# Autodesk Inventor assembly: 1. Prototype Plate Assembly
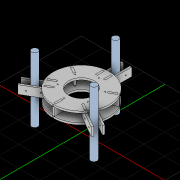
[picture p0: Inventor's stored thumbnail of the model, 180x180]
Saved by Autodesk Inventor 2020.1 (Build 241239000, 239)
## iProperties
Created: 2019-08-27
Part Number: 1. Prototype Plate Assembly
Document SubType Name: Assembly
Designer: Oliver Frolovs
Mass: 1152 g
Surface Area: 3223.44 cm^2
Volume: 1152 cm^3
Density: 1 g/cm^3
Author: Oliver Frolovs
## Documents named in this file (6)
- C:\Users\of12343\Documents\Projects\prototype-plate\1. Prototype Plate Assembly.iam
- C:\Users\of12343\Documents\Projects\prototype-plate\Prototype Plate Base.ipt
- C:\Users\of12343\Documents\Projects\prototype-plate\Inner Rib.ipt
- C:\Users\of12343\Documents\Projects\prototype-plate\0. All Parameters.ipt
- C:\Users\of12343\Documents\Projects\prototype-plate\Outer Rib.ipt
- C:\Users\of12343\Documents\Projects\prototype-plate\Locate Rig Columns.ipt
## Components (12 placed, 4 different names)
1. Prototype Plate Base:1 — Rigid:3, Rigid:4, Rigid:5, Rigid:6
2. Prototype Plate Base:2 — Rigid:4
3. Locate Rig Columns:1 — Flush:1
4. Inner Rib — Rigid:3
5. Inner Rib:2
6. Inner Rib:3
7. Outer Rib:1 — Rigid:5
8. Outer Rib:2 — Rigid:6
9. Outer Rib:3
10. Outer Rib:4
11. Outer Rib:5
12. Outer Rib:6
## Component patterns: Inner Ribs (3 elements), Outer Ribs (3 elements)
## Relationships (5: WeldJoint 4, Flush 1)
- Rigid:3 [WeldJoint]: Prototype Plate Base:1 ↔ Inner Rib
- Rigid:4 [WeldJoint] (40 mm): Prototype Plate Base:1 ↔ Prototype Plate Base:2
- Rigid:5 [WeldJoint]: Prototype Plate Base:1 ↔ Outer Rib:1
- Rigid:6 [WeldJoint]: Prototype Plate Base:1 ↔ Outer Rib:2
- Flush:1: Locate Rig Columns:1
## Named parameters: InnerRibHeight = 40 mm, RigColumnsPCD = 328 mm, RigColumnsDiameter = 30 mm
